# Autodesk Inventor assembly: 002 - Крепление СБ
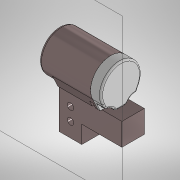
[picture p0: Inventor's stored thumbnail of the model, 180x180]
Saved by Autodesk Inventor 2022 (Build 260153000, 153)
## iProperties
Created: 2022-01-16
Part Number: 002 - Крепление СБ
Document SubType Name: Assembly
Designer: Петров Иван
Author: Петров Иван
## Documents named in this file (4)
- E:\IVAN\Ivan_desktop\Kvantorium\Projects\YouBotRobot\design\002 - Крепление СБ.iam
- E:\IVAN\Ivan_desktop\Kvantorium\Projects\YouBotRobot\design\standart_components\dc_gear_motor_12V_500rpm.ipt
- E:\IVAN\Ivan_desktop\Kvantorium\Projects\YouBotRobot\design\002-001 - Крепление.ipt
- E:\IVAN\Ivan_desktop\Kvantorium\Projects\YouBotRobot\design\002-002 - Крышка мотора.ipt
## Components (3 placed, 3 different names)
1. dc_gear_motor_12V_500rpm:1 — Совмещение:1, Совмещение:2, Совмещение:3
2. 002-001 - Крепление:1 — Совмещение:1, Совмещение:2, Совмещение:3, Совмещение:5, Совмещение:6, Совмещение:7
3. 002-002 - Крышка мотора:1 — Совмещение:5, Совмещение:6, Совмещение:7
## Relationships (6: Mate 6)
- Совмещение:1 [Mate]: dc_gear_motor_12V_500rpm:1 ↔ 002-001 - Крепление:1
- Совмещение:2 [Mate]: dc_gear_motor_12V_500rpm:1 ↔ 002-001 - Крепление:1
- Совмещение:3 [Mate]: dc_gear_motor_12V_500rpm:1 ↔ 002-001 - Крепление:1
- Совмещение:5 [Mate]: 002-001 - Крепление:1 ↔ 002-002 - Крышка мотора:1
- Совмещение:6 [Mate]: 002-001 - Крепление:1 ↔ 002-002 - Крышка мотора:1
- Совмещение:7 [Mate]: 002-001 - Крепление:1 ↔ 002-002 - Крышка мотора:1
